# Autodesk Inventor assembly: Press_Assembly
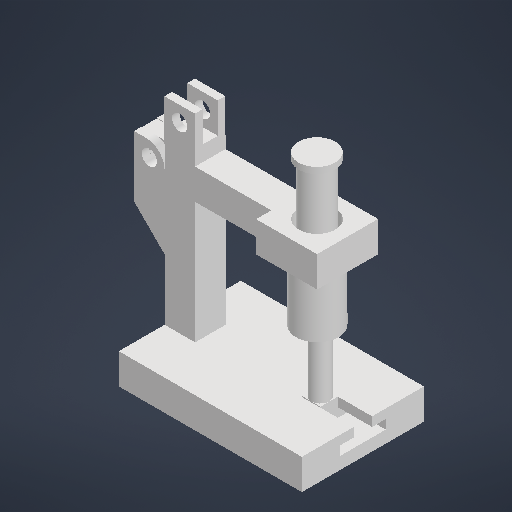
[picture p0: Inventor's stored thumbnail of the model, 512x512]
Saved by Autodesk Inventor 2026.1 (Build 301233020, 233B)
## iProperties
Created: 2025-09-29
Part Number: Press_Assembly
Document SubType Name: Assembly
Designer: Gamec
Author: Gamec
## Documents named in this file (5)
- C:\Users\Gamec\OneDrive\Desktop\USCRC\Projects\AcidBaseRockets\Press\Press_Assembly.iam
- C:\Users\Gamec\OneDrive\Desktop\USCRC\Projects\AcidBaseRockets\Press\Press_Base.ipt
- C:\Users\Gamec\OneDrive\Desktop\USCRC\Projects\AcidBaseRockets\Press\Press_Lower_Arm.ipt
- C:\Users\Gamec\OneDrive\Desktop\USCRC\Projects\AcidBaseRockets\Press\Press_Head.ipt
- C:\Users\Gamec\OneDrive\Desktop\USCRC\Projects\AcidBaseRockets\Press\Press_Mandrel.ipt
## Components (4 placed, 4 different names)
1. Press_Base:1 — Rotational:1, Mate:1, Mate:2, Mate:3
2. Press_Lower_Arm:1 — Rotational:1, Cylindrical:1
3. Press_Head:1 — Cylindrical:1
4. Press_Mandrel:1 — Mate:1, Mate:2, Mate:3
## Relationships (5: Mate 3, RevoluteJoint 1, CylindricalJoint 1)
- Rotational:1 [RevoluteJoint] (0.0635 mm): Press_Base:1 ↔ Press_Lower_Arm:1
- Cylindrical:1: Press_Lower_Arm:1 ↔ Press_Head:1
- Mate:1: Press_Base:1 ↔ Press_Mandrel:1
- Mate:2: Press_Base:1 ↔ Press_Mandrel:1
- Mate:3 (0.127 mm): Press_Base:1 ↔ Press_Mandrel:1
